# Autodesk Inventor assembly: Motor+ArmToBottom
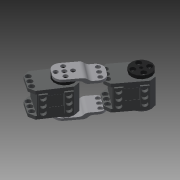
[picture p0: Inventor's stored thumbnail of the model, 180x180]
Saved by Autodesk Inventor 2014 (Build 180170000, 170)
## iProperties
Created: 2014-03-07
Part Number: Motor+ArmToBottom
Document SubType Name: Assembly
Designer: Grégoire
Author: Grégoire
## Documents named in this file (5)
- C:\Users\Bless\Desktop\XL320\src\Motor+ArmToBottom.iam
- C:\Users\Bless\Desktop\XL320\src\Motor.ipt
- C:\Users\Bless\Desktop\XL320\src\Arm.ipt
- C:\Users\Bless\Desktop\XL320\src\CounterArm.ipt
- C:\Users\Bless\Desktop\XL320\src\ArmToBottom.ipt
## Components (8 placed, 4 different names)
1. Motor:1 — Placage:1, Placage:2, Placage:3, Placage:4
2. Arm:1 — Placage:3, Placage:4, Placage:15, Placage:16, Placage:17
3. CounterArm:1 — Placage:1, Placage:2, Placage:9, Placage:10, Placage:11
4. Motor:2 — Placage:12, Placage:13, Placage:14, Placage:18
5. Arm:2
6. CounterArm:2
7. ArmToBottom:1 — Placage:9, Placage:10, Placage:11, Placage:12, Placage:13, Placage:14
8. ArmToBottom:2 — Placage:15, Placage:16, Placage:17, Placage:18
## Relationships (18: Mate 18)
- Placage:1 [Mate]: Motor:1 ↔ CounterArm:1
- Placage:2 [Mate]: Motor:1 ↔ CounterArm:1
- Placage:3 [Mate]: Motor:1 ↔ Arm:1
- Placage:4 [Mate]: Motor:1 ↔ Arm:1
- [Mate]: Motor:2 ↔ CounterArm:2
- [Mate]: Motor:2 ↔ CounterArm:2
- [Mate]: Motor:2 ↔ Arm:2
- [Mate]: Motor:2 ↔ Arm:2
- Placage:9 [Mate]: CounterArm:1 ↔ ArmToBottom:1
- Placage:10 [Mate]: CounterArm:1 ↔ ArmToBottom:1
- Placage:11 [Mate]: CounterArm:1 ↔ ArmToBottom:1
- Placage:12 [Mate]: Motor:2 ↔ ArmToBottom:1
- Placage:13 [Mate]: Motor:2 ↔ ArmToBottom:1
- Placage:14 [Mate]: Motor:2 ↔ ArmToBottom:1
- Placage:15 [Mate]: Arm:1 ↔ ArmToBottom:2
- Placage:16 [Mate]: Arm:1 ↔ ArmToBottom:2
- Placage:17 [Mate]: Arm:1 ↔ ArmToBottom:2
- Placage:18 [Mate]: Motor:2 ↔ ArmToBottom:2
## Named parameters: d4_d0 = 0 mm, d5_d1 = 0 mm, d6_d2 = 0 mm, d7_d3 = 0 mm
